# Autodesk Inventor assembly: CL3-100
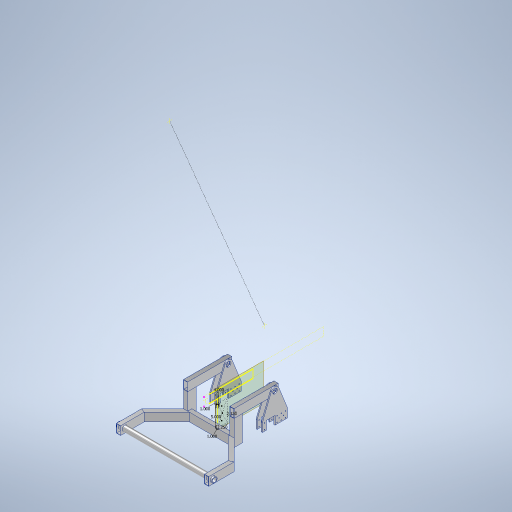
[picture p0: Inventor's stored thumbnail of the model, 512x512]
Saved by Autodesk Inventor 2023.4 (Build 274418000, 418)
## iProperties
Created: 2025-01-28
Part Number: CL3-100
Document SubType Name: Assembly
Designer: slick
Mass: 5241.21 g
Surface Area: 12801.1 cm^2
Volume: 1941.19 cm^3
Density: 2.7 g/cm^3
Author: slick
## Documents named in this file (9)
- C:\Users\mavericks\Documents\GitHub\2025-ReefScape---CAD\Climber\CL3\CL3-100.iam
- C:\Users\mavericks\Documents\GitHub\2025-ReefScape---CAD\Climber\CL3\CL3-001.ipt
- C:\Users\mavericks\Documents\GitHub\2025-ReefScape---CAD\Climber\CL3\CL3-002.ipt
- C:\Users\mavericks\Documents\GitHub\2025-ReefScape---CAD\Climber\CL3\CL3-003.ipt
- C:\Users\mavericks\Documents\GitHub\2025-ReefScape---CAD\Climber\CL3\CL3-004.ipt
- C:\Users\mavericks\Documents\GitHub\2025-ReefScape---CAD\Climber\CL3\CL3-005.ipt
- C:\Users\mavericks\Documents\GitHub\2025-ReefScape---CAD\Climber\CL3\CL3-006.ipt
- C:\Users\mavericks\Documents\GitHub\2025-ReefScape---CAD\Field Items\Full Field\FE-2025\GE-25201.iam
- C:\Users\mavericks\Documents\GitHub\2025-ReefScape---CAD\Climber\CL3\CL3-007.ipt
## Components (15 placed, 8 different names)
1. CL3-001:1 — Mate:9, Flush:5, Mate:10, Mate:11, Mate:15, Mate:16, Symmetry:1, Angle:1, Mate:22, Flush:14
2. CL3-002:1 — Flush:2, Mate:3, Mate:4, Mate:26, Flush:19, Mate:28
3. CL3-003:1 — Flush:2, Mate:3, Mate:4, Mate:19
4. CL3-001:2 — Mate:9, Flush:5, Mate:13, Mate:14, Mate:17, Symmetry:1, Mate:23, Flush:13
5. CL3-002:2 — Mate:27, Flush:20, Mate:29
6. CL3-003:2
7. CL3-004:1 — Flush:7, Mate:12, Mate:13, Flush:9, Mate:17
8. CL3-004:2 — Flush:7, Mate:10, Mate:15, Flush:8
9. CL3-004:3 — Mate:11, Mate:16, Flush:8, Angle:1, Symmetry:2, Mate:24
10. CL3-004:4 — Mate:12, Mate:14, Flush:9, Symmetry:2
11. CL3-005:1 — Tangent:2, Mate:25, Flush:16, Flush:18
12. CL3-006:1 — Mate:19, Tangent:1, Mate:21
13. GE-25201:1 [sub-assembly] — Mate:20, Tangent:1, Tangent:2, Mate:21
14. CL3-007:1 — Mate:22, Flush:14, Flush:15, Mate:24, Mate:25, Flush:16, Mate:26, Flush:19, Mate:28
15. CL3-007:2 — Mate:23, Flush:13, Flush:15, Flush:18, Mate:27, Flush:20, Mate:29
## Relationships (42: Mate 24, Flush 13, Symmetry 2, Tangent 2, Angle 1)
- Flush:2: CL3-002:1 ↔ CL3-003:1
- Mate:3: CL3-002:1 ↔ CL3-003:1
- Mate:4: CL3-002:1 ↔ CL3-003:1
- [Flush]: CL3-002:2 ↔ CL3-003:2
- [Mate]: CL3-002:2 ↔ CL3-003:2
- [Mate]: CL3-002:2 ↔ CL3-003:2
- Mate:9 (254 mm): CL3-001:1 ↔ CL3-001:2
- Flush:5: CL3-001:1 ↔ CL3-001:2
- Flush:7: CL3-004:1 ↔ CL3-004:2
- Mate:10: CL3-001:1 ↔ CL3-004:2
- Mate:11: CL3-001:1 ↔ CL3-004:3
- Mate:12: CL3-004:1 ↔ CL3-004:4
- Mate:13: CL3-001:2 ↔ CL3-004:1
- Mate:14: CL3-001:2 ↔ CL3-004:4
- Mate:15: CL3-001:1 ↔ CL3-004:2
- Mate:16: CL3-001:1 ↔ CL3-004:3
- Flush:8: CL3-004:2 ↔ CL3-004:3
- Flush:9: CL3-004:1 ↔ CL3-004:4
- Mate:17: CL3-001:2 ↔ CL3-004:1
- Mate:19: CL3-003:1 ↔ CL3-006:1
- Symmetry:1: CL3-001:1 ↔ CL3-001:2
- Mate:20: GE-25201:1
- Tangent:1: CL3-006:1 ↔ GE-25201:1
- Tangent:2: CL3-005:1 ↔ GE-25201:1
- Mate:21 (-76.2 mm): CL3-006:1 ↔ GE-25201:1
- Angle:1 (90 deg): CL3-001:1 ↔ CL3-004:3
- Symmetry:2: CL3-004:3 ↔ CL3-004:4
- Mate:22: CL3-001:1 ↔ CL3-007:1
- Mate:23: CL3-001:2 ↔ CL3-007:2
- Flush:13: CL3-001:2 ↔ CL3-007:2
- Flush:14: CL3-001:1 ↔ CL3-007:1
- Flush:15: CL3-007:1 ↔ CL3-007:2
- Mate:24 (113.792 mm): CL3-004:3 ↔ CL3-007:1
- Mate:25: CL3-005:1 ↔ CL3-007:1
- Flush:16: CL3-005:1 ↔ CL3-007:1
- Flush:18: CL3-005:1 ↔ CL3-007:2
- Mate:26: CL3-002:1 ↔ CL3-007:1
- Flush:19: CL3-002:1 ↔ CL3-007:1
- Mate:27: CL3-002:2 ↔ CL3-007:2
- Flush:20: CL3-002:2 ↔ CL3-007:2
- Mate:28: CL3-002:1 ↔ CL3-007:1
- Mate:29: CL3-002:2 ↔ CL3-007:2
## Named parameters: d27_d21 = 0 mm, d28_d22 = 0 mm, d29_d23 = 0 mm
